# Autodesk Inventor assembly: 可删
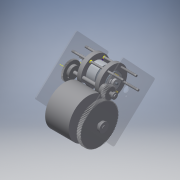
[picture p0: Inventor's stored thumbnail of the model, 180x180]
Saved by Autodesk Inventor 2019 (Build 230136000, 136)
## iProperties
Created: 2020-09-26
Part Number: 可删
Material: 一般
Document SubType Name: Assembly
Designer: zhept
Author: zhept
## Documents named in this file (16)
- C:\Users\zhept\OneDrive\大学\rrst\足回り2020\可删.iam
- C:\Users\zhept\OneDrive\大学\rrst\足回り2020\KHK_SS0590AOn\KHK_SS0590AOn.ipt
- C:\Users\zhept\OneDrive\大学\rrst\足回り2020\KHK_SS0530BOn\KHK_SS0530BOn.ipt
- C:\Users\zhept\OneDrive\大学\rrst\RS775\モーター\モーター RS775-8513DF.iam
- C:\Users\zhept\OneDrive\大学\rrst\足回り2020\足回り製作中.iam
- C:\Users\zhept\OneDrive\大学\rrst\足回り2020\KHK_SS128On\KHK_SS128On.ipt
- C:\Users\zhept\OneDrive\大学\rrst\足回り2020\KHK_SS196On\KHK_SS196On.ipt
- C:\Users\zhept\OneDrive\大学\rrst\足回り2020\円 46.9mm\円 46.9mm.ipt
- C:\Users\zhept\OneDrive\大学\rrst\足回り2020\六角スペーサー\六角スペーサー.ipt
- C:\Users\zhept\OneDrive\大学\rrst\足回り2020\円 42.5mm\円 42.5mm.ipt
- C:\Users\zhept\OneDrive\大学\rrst\足回り2020\板.ipt
- C:\Users\zhept\OneDrive\大学\rrst\玉軸受1 F605ZZ\玉軸受1 F605ZZ.ipt
- C:\Users\zhept\OneDrive\大学\rrst\玉軸受2 F608ZZ\玉軸受2 F608ZZ.ipt
- C:\Users\zhept\OneDrive\大学\rrst\足回り2020\円柱5mm.ipt
- C:\Users\zhept\OneDrive\大学\rrst\足回り2020\円柱8mm.ipt
- C:\Users\zhept\OneDrive\大学\rrst\足回り2020\円柱10mm.ipt
## Components (21 placed, 15 different names)
1. KHK_SS0590AOn:1 — フラッシュ:1, フラッシュ:3, メイト:2
2. KHK_SS0530BOn:1 — フラッシュ:2, フラッシュ:3, メイト:1, 回転:1
3. モーター RS775-8513DF:1 [sub-assembly] — 回転:1, メイト:9, 回転:2, 回転:3, メイト:10
4. 足回り製作中:1 [sub-assembly] — 挿入:1
5. KHK_SS128On:1 — メイト:4, フラッシュ:4, フラッシュ:6
6. KHK_SS196On:1 — 挿入:1, フラッシュ:5, フラッシュ:6, メイト:6
7. 円 46.9mm:1 — メイト:9, 挿入:5, メイト:12
8. 六角スペーサー:1 — 回転:3, 挿入:2
9. 六角スペーサー:2 — 回転:2, 挿入:3
10. 円 42.5mm:1 — メイト:10, 挿入:5
11. 板:1 — 挿入:2, 挿入:3, 挿入:4, 角度:1, メイト:12, 回転:4, 回転:5, 挿入:6, 挿入:7, 挿入:8
12. 板:2 — 挿入:4, 角度:1, リジッド:1, 回転:6
13. 玉軸受1 F605ZZ:1 — 回転:5, 挿入:9
14. 玉軸受1 F605ZZ:2 — 回転:6
15. 玉軸受2 F608ZZ:1 — リジッド:1
16. 玉軸受2 F608ZZ:2 — 回転:4, 挿入:10
17. 円柱5mm:1 — 挿入:6
18. 円柱5mm:2 — 挿入:8
19. 円柱5mm:3 — 挿入:7
20. 円柱8mm:1 — 挿入:9
21. 円柱10mm:1 — 挿入:10
## Relationships (34: Mate 10, Insert 10, Flush 6, RevoluteJoint 6, Angle 1, WeldJoint 1)
- フラッシュ:1 [Flush]: KHK_SS0590AOn:1
- フラッシュ:2 [Flush]: KHK_SS0530BOn:1
- フラッシュ:3 [Flush]: KHK_SS0590AOn:1 ↔ KHK_SS0530BOn:1
- メイト:1 [Mate]: KHK_SS0530BOn:1
- メイト:2 [Mate]: KHK_SS0590AOn:1
- メイト:3 [Mate] (30 mm)
- 回転:1 [RevoluteJoint]: KHK_SS0530BOn:1 ↔ モーター RS775-8513DF:1
- メイト:4 [Mate]: KHK_SS128On:1
- メイト:5 [Mate]
- 挿入:1 [Insert]: 足回り製作中:1 ↔ KHK_SS196On:1
- フラッシュ:4 [Flush]: KHK_SS128On:1
- フラッシュ:5 [Flush]: KHK_SS196On:1
- フラッシュ:6 [Flush]: KHK_SS128On:1 ↔ KHK_SS196On:1
- メイト:6 [Mate]: KHK_SS196On:1
- メイト:7 [Mate] (62 mm)
- メイト:9 [Mate]: モーター RS775-8513DF:1 ↔ 円 46.9mm:1
- 回転:2 [RevoluteJoint]: モーター RS775-8513DF:1 ↔ 六角スペーサー:2
- 回転:3 [RevoluteJoint]: モーター RS775-8513DF:1 ↔ 六角スペーサー:1
- メイト:10 [Mate]: モーター RS775-8513DF:1 ↔ 円 42.5mm:1
- 挿入:2 [Insert]: 六角スペーサー:1 ↔ 板:1
- 挿入:3 [Insert]: 六角スペーサー:2 ↔ 板:1
- 挿入:4 [Insert] (115 mm): 板:1 ↔ 板:2
- 角度:1 [Angle] (0 deg): 板:1 ↔ 板:2
- 挿入:5 [Insert] (45 mm): 円 46.9mm:1 ↔ 円 42.5mm:1
- メイト:12 [Mate] (28.5 mm): 円 46.9mm:1 ↔ 板:1
- 回転:4 [RevoluteJoint]: 板:1 ↔ 玉軸受2 F608ZZ:2
- リジッド:1 [WeldJoint]: 板:2 ↔ 玉軸受2 F608ZZ:1
- 回転:5 [RevoluteJoint]: 板:1 ↔ 玉軸受1 F605ZZ:1
- 回転:6 [RevoluteJoint]: 板:2 ↔ 玉軸受1 F605ZZ:2
- 挿入:6 [Insert] (-5 mm): 板:1 ↔ 円柱5mm:1
- 挿入:7 [Insert] (-5 mm): 板:1 ↔ 円柱5mm:3
- 挿入:8 [Insert] (-5 mm): 板:1 ↔ 円柱5mm:2
- 挿入:9 [Insert] (-5 mm): 玉軸受1 F605ZZ:1 ↔ 円柱8mm:1
- 挿入:10 [Insert] (-5 mm): 玉軸受2 F608ZZ:2 ↔ 円柱10mm:1
